(part 1 of 2)
# Autodesk Inventor assembly: Top_Backboard Assy
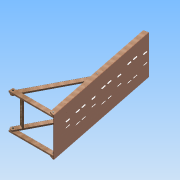
[picture p0: Inventor's stored thumbnail of the model, 180x180]
Saved by Autodesk Inventor 2018.1 (Build 221171000, 171)
## iProperties
Created: 2019-03-15
Part Number: Top_Backboard Assy
Document SubType Name: Assembly
Designer: James
Author: James
## Documents named in this file (20)
- C:\Users\admin\Desktop\Ball-Machine\Top Level\Top_Backboard Assy.iam
- C:\Users\admin\Desktop\Ball-Machine\Top Level\Top_Backboard.ipt
- C:\Users\admin\Desktop\Ball-Machine\Top Level\Top_Reinforcement 2.ipt
- C:\Users\admin\Desktop\Ball-Machine\Top Level\Top_Reinforcement_LHS.ipt
- C:\Users\admin\Desktop\Ball-Machine\Top Level\Top_Reinforcement_RHS.ipt
- C:\Users\admin\Desktop\Ball-Machine\Top Level\Din97 - 8x80 - Steel Wood Screw.ipt
- C:\Users\admin\Desktop\Ball-Machine\Top Level\Top_Hinge Cylinder.ipt
- C:\Users\admin\Desktop\Ball-Machine\Top Level\Top_Hinge End.ipt
- C:\Users\admin\Desktop\Ball-Machine\Top Level\Socket Cap Screw - Standard - (A2) - M8 x 20.ipt
- C:\Users\admin\Desktop\Ball-Machine\Top Level\Top_Floor Plank.ipt
- C:\Users\admin\Desktop\Ball-Machine\Top Level\Top_Reinforcement 3.ipt
- C:\Users\admin\Desktop\Ball-Machine\Top Level\Top_Rear Plank_RHS.ipt
- C:\Users\admin\Desktop\Ball-Machine\Top Level\Top_Rear Plank_LHS.ipt
- C:\Users\admin\Desktop\Ball-Machine\Top Level\Top_Spacer.ipt
- C:\Users\admin\Desktop\Ball-Machine\Top Level\Top_Hinge Cylinder Long.ipt
- C:\Users\admin\Desktop\Ball-Machine\Top Level\Top_Angle Bracket.ipt
- C:\Users\admin\Desktop\Ball-Machine\Selection Sort\Nyloc Nut - M4.ipt
- C:\Users\admin\Desktop\Ball-Machine\Selection Sort\Socket Cap Screw - Standard - (A2) - M4 x 16.ipt
- C:\Users\admin\Desktop\Ball-Machine\Top Level\Socket Cap Screw - Standard - (A2) - M4 x 25.ipt
- C:\Users\admin\Desktop\Ball-Machine\Top Level\Din97 - 4x25 - Steel Wood Screw.ipt
## Components (264 placed, 19 different names)
1. Top_Backboard:1 — Flush:3, Mate:1, Mate:2, Flush:5, Flush:6, Flush:7, Flush:8, Flush:10, Mate:5, Mate:320, Mate:321, Mate:322, Mate:323, Mate:324, Mate:325, Mate:326, Mate:327, Mate:328, Mate:329, Mate:330, Mate:331, Mate:332, Mate:333, Mate:334, Mate:335, Mate:336, Mate:337, Mate:338, Mate:339, Mate:340, Mate:341, Mate:342, Mate:343, Mate:344, Mate:345, Mate:346, Mate:347, Mate:348, Mate:349, Mate:350, Mate:351, Mate:352, Mate:353, Mate:354, Mate:355, Mate:356, Mate:357, Mate:358, Mate:359, Mate:360, Mate:361, Mate:362, Mate:363, Mate:364, Mate:365, Mate:366, Mate:367, Flush:29, Mate:368, Flush:30, Mate:369, Mate:370, Mate:371, Flush:31, Flush:32, Flush:33
2. Top_Reinforcement_LHS:1 — Mate:1, Flush:4, Flush:5, Flush:6, Flush:10, Mate:3, Mate:6, Mate:7, Mate:12, Mate:13, Flush:12, Mate:14, Mate:15, Mate:20, Mate:23, Mate:32, Mate:73, Mate:74, Mate:75, Mate:76, Mate:77, Mate:89, Mate:90, Mate:362
3. Top_Reinforcement_RHS:1 — Mate:2, Flush:4, Flush:7, Flush:8, Mate:4, Mate:8, Mate:9, Mate:10, Mate:11, Flush:13, Mate:21, Mate:22, Mate:31, Mate:55, Mate:56, Mate:64, Mate:65, Mate:66, Mate:67, Mate:68, Mate:82, Mate:83, Mate:363
4. Top_Floor Plank:1 — Mate:21, Mate:22, Flush:15, Mate:29, Mate:30, Mate:57, Mate:58, Mate:59
5. Top_Floor Plank:2 — Mate:20, Mate:23, Flush:15, Mate:24, Mate:25, Mate:26, Mate:27, Mate:28, Mate:61, Mate:62
6. Top_Rear Plank_RHS:1 — Mate:29, Mate:30, Flush:16, Mate:31, Mate:36, Mate:37, Mate:38, Mate:41, Mate:42, Flush:17, Mate:60, Mate:84, Mate:85
7. Top_Rear Plank_LHS:1 — Mate:27, Mate:28, Flush:16, Mate:32, Mate:33, Mate:34, Mate:35, Mate:39, Mate:40, Flush:20, Mate:63, Mate:91
8. Top_Reinforcement 3:1 — Mate:33, Mate:34, Mate:35, Mate:36, Mate:37, Mate:38
9. Top_Spacer:1 — Mate:64, Mate:65, Mate:66, Mate:67, Mate:68, Mate:69, Mate:70, Mate:71, Mate:72, Flush:24
10. Top_Spacer:2 — Mate:73, Mate:74, Mate:75, Mate:76, Mate:77, Flush:28, Mate:78, Mate:79, Mate:80, Mate:81
11. Top_Hinge End:6 — Mate:91, Mate:92, Mate:93, Mate:94, Mate:95
12. Top_Hinge Cylinder Long:2 — Mate:89, Mate:90, Mate:92, Mate:93
13. Din97 - 8x80 - Steel Wood Screw:17 — Mate:69, Flush:21
14. Din97 - 8x80 - Steel Wood Screw:18 — Mate:70, Flush:21, Flush:22, Flush:23, Flush:24
15. Din97 - 8x80 - Steel Wood Screw:19 — Mate:71, Flush:23
16. Din97 - 8x80 - Steel Wood Screw:20 — Mate:72, Flush:22
17. Din97 - 8x80 - Steel Wood Screw:21 — Flush:25, Flush:26, Flush:27, Flush:28, Mate:78
18. Din97 - 8x80 - Steel Wood Screw:22 — Flush:25, Mate:79
19. Din97 - 8x80 - Steel Wood Screw:23 — Flush:26, Mate:80
20. Din97 - 8x80 - Steel Wood Screw:24 — Flush:27, Mate:81
21. Socket Cap Screw - Standard - (A2) - M8 x 20:5 — Mate:87, Mate:88
22. Top_Hinge Cylinder Long:1 — Mate:82, Mate:83, Mate:86
23. Top_Hinge End:5 — Mate:84, Mate:85, Mate:86, Mate:87, Mate:88
24. Socket Cap Screw - Standard - (A2) - M8 x 20:6 — Mate:94, Mate:95
25. Socket Cap Screw - Standard - (A2) - M8 x 20:4
26. Top_Hinge End:4 — Mate:57
27. Top_Hinge Cylinder:4 — Mate:55, Mate:56
28. Socket Cap Screw - Standard - (A2) - M8 x 20:3
29. Top_Hinge End:3 — Mate:60
30. Top_Hinge Cylinder:3 — Mate:58, Mate:59
31. Socket Cap Screw - Standard - (A2) - M8 x 20:2
32. Top_Hinge End:2 — Mate:63
33. Top_Hinge Cylinder:2 — Mate:61, Mate:62
34. Din97 - 8x80 - Steel Wood Screw:16 — Mate:41, Flush:18
35. Din97 - 8x80 - Steel Wood Screw:15 — Mate:42, Flush:17, Flush:18
36. Din97 - 8x80 - Steel Wood Screw:14 — Mate:40, Flush:19, Flush:20
37. Din97 - 8x80 - Steel Wood Screw:13 — Mate:39, Flush:19
38. Socket Cap Screw - Standard - (A2) - M8 x 20:1 — Mate:18, Mate:19
39. Top_Hinge End:1 — Mate:16, Mate:17, Mate:18, Mate:19, Mate:26
40. Top_Hinge Cylinder:1 — Mate:14, Mate:15, Mate:16, Mate:17
41. Top_Angle Bracket:1 — Mate:104, Mate:105, Mate:106, Mate:107, Mate:108, Mate:109, Mate:110, Mate:111, Mate:320
42. Nyloc Nut - M4:1 — Mate:100
43. Nyloc Nut - M4:2 — Mate:103
44. Nyloc Nut - M4:3 — Mate:102
45. Socket Cap Screw - Standard - (A2) - M4 x 16:1 — Mate:102, Mate:108, Mate:110
46. Nyloc Nut - M4:4 — Mate:101
47. Socket Cap Screw - Standard - (A2) - M4 x 16:2 — Mate:101, Mate:109, Mate:111
48. Socket Cap Screw - Standard - (A2) - M4 x 25:1 — Mate:100, Mate:106, Mate:107, Mate:321
49. Socket Cap Screw - Standard - (A2) - M4 x 25:2 — Mate:103, Mate:104, Mate:105, Mate:322
50. Top_Angle Bracket:2 — Mate:323
51. Nyloc Nut - M4:5
52. Nyloc Nut - M4:6
53. Nyloc Nut - M4:7
54. Socket Cap Screw - Standard - (A2) - M4 x 16:3
55. Nyloc Nut - M4:8
56. Socket Cap Screw - Standard - (A2) - M4 x 16:4
57. Socket Cap Screw - Standard - (A2) - M4 x 25:3 — Mate:336
58. Socket Cap Screw - Standard - (A2) - M4 x 25:4 — Mate:337
59. Top_Angle Bracket:3 — Mate:324
60. Nyloc Nut - M4:9
61. Nyloc Nut - M4:10
62. Nyloc Nut - M4:11
63. Socket Cap Screw - Standard - (A2) - M4 x 16:5
64. Nyloc Nut - M4:12
65. Socket Cap Screw - Standard - (A2) - M4 x 16:6
66. Socket Cap Screw - Standard - (A2) - M4 x 25:5 — Mate:338
67. Socket Cap Screw - Standard - (A2) - M4 x 25:6 — Mate:339
68. Top_Angle Bracket:4 — Mate:325
69. Nyloc Nut - M4:13
70. Nyloc Nut - M4:14
71. Nyloc Nut - M4:15
72. Socket Cap Screw - Standard - (A2) - M4 x 16:7
73. Nyloc Nut - M4:16
74. Socket Cap Screw - Standard - (A2) - M4 x 16:8
75. Socket Cap Screw - Standard - (A2) - M4 x 25:7 — Mate:340
76. Socket Cap Screw - Standard - (A2) - M4 x 25:8 — Mate:341
77. Top_Angle Bracket:5 — Mate:326
78. Nyloc Nut - M4:17
79. Nyloc Nut - M4:18
80. Nyloc Nut - M4:19
81. Socket Cap Screw - Standard - (A2) - M4 x 16:9
82. Nyloc Nut - M4:20
83. Socket Cap Screw - Standard - (A2) - M4 x 16:10
84. Socket Cap Screw - Standard - (A2) - M4 x 25:9 — Mate:342
85. Socket Cap Screw - Standard - (A2) - M4 x 25:10 — Mate:343
86. Top_Angle Bracket:6 — Mate:327
87. Nyloc Nut - M4:21
88. Nyloc Nut - M4:22
89. Nyloc Nut - M4:23
90. Socket Cap Screw - Standard - (A2) - M4 x 16:11
91. Nyloc Nut - M4:24
92. Socket Cap Screw - Standard - (A2) - M4 x 16:12
93. Socket Cap Screw - Standard - (A2) - M4 x 25:11 — Mate:344
94. Socket Cap Screw - Standard - (A2) - M4 x 25:12 — Mate:345
95. Top_Angle Bracket:7 — Mate:328
96. Nyloc Nut - M4:25
97. Nyloc Nut - M4:26
98. Nyloc Nut - M4:27
99. Socket Cap Screw - Standard - (A2) - M4 x 16:13
100. Nyloc Nut - M4:28
101. Socket Cap Screw - Standard - (A2) - M4 x 16:14
102. Socket Cap Screw - Standard - (A2) - M4 x 25:13 — Mate:348
103. Socket Cap Screw - Standard - (A2) - M4 x 25:14 — Mate:349
104. Top_Angle Bracket:12 — Mate:333
105. Nyloc Nut - M4:45
106. Nyloc Nut - M4:46
107. Nyloc Nut - M4:47
108. Socket Cap Screw - Standard - (A2) - M4 x 16:23
109. Nyloc Nut - M4:48
110. Socket Cap Screw - Standard - (A2) - M4 x 16:24
111. Socket Cap Screw - Standard - (A2) - M4 x 25:23 — Mate:346
112. Socket Cap Screw - Standard - (A2) - M4 x 25:24 — Mate:347
113. Top_Reinforcement 2:1 — Mate:3, Mate:4, Mate:5, Mate:6, Mate:7, Mate:8, Mate:9, Mate:366
114. Din97 - 8x80 - Steel Wood Screw:1 — Mate:10, Flush:13, Flush:14
115. Din97 - 8x80 - Steel Wood Screw:2 — Mate:11, Flush:14
116. Din97 - 8x80 - Steel Wood Screw:3 — Mate:12, Flush:11, Flush:12
117. Din97 - 8x80 - Steel Wood Screw:4 — Mate:13, Flush:11
118. Top_Reinforcement 2:2 — Mate:364
119. Din97 - 8x80 - Steel Wood Screw:5
120. Din97 - 8x80 - Steel Wood Screw:6
121. Din97 - 8x80 - Steel Wood Screw:7
122. Din97 - 8x80 - Steel Wood Screw:8
123. Top_Reinforcement 2:3 — Mate:365
124. Din97 - 8x80 - Steel Wood Screw:9
125. Din97 - 8x80 - Steel Wood Screw:10
126. Din97 - 8x80 - Steel Wood Screw:11
127. Din97 - 8x80 - Steel Wood Screw:12
128. Top_Angle Bracket:14 — Mate:335
129. Socket Cap Screw - Standard - (A2) - M4 x 16:27
130. Socket Cap Screw - Standard - (A2) - M4 x 25:28 — Mate:361
131. Nyloc Nut - M4:55
132. Socket Cap Screw - Standard - (A2) - M4 x 16:28
133. Socket Cap Screw - Standard - (A2) - M4 x 25:27 — Mate:360
134. Nyloc Nut - M4:56
135. Nyloc Nut - M4:52
136. Socket Cap Screw - Standard - (A2) - M4 x 16:26
137. Socket Cap Screw - Standard - (A2) - M4 x 25:25 — Mate:358
138. Top_Angle Bracket:13 — Mate:334
139. Nyloc Nut - M4:51
140. Socket Cap Screw - Standard - (A2) - M4 x 16:25
141. Socket Cap Screw - Standard - (A2) - M4 x 25:26 — Mate:359
142. Socket Cap Screw - Standard - (A2) - M4 x 25:18 — Mate:353
143. Socket Cap Screw - Standard - (A2) - M4 x 16:17
144. Top_Angle Bracket:9 — Mate:330
145. Nyloc Nut - M4:35
146. Socket Cap Screw - Standard - (A2) - M4 x 25:17 — Mate:352
147. Socket Cap Screw - Standard - (A2) - M4 x 16:18
148. Nyloc Nut - M4:36
149. Nyloc Nut - M4:32
150. Socket Cap Screw - Standard - (A2) - M4 x 16:16
151. Socket Cap Screw - Standard - (A2) - M4 x 25:15 — Mate:350
152. Top_Angle Bracket:8 — Mate:329
153. Nyloc Nut - M4:31
154. Socket Cap Screw - Standard - (A2) - M4 x 16:15
155. Socket Cap Screw - Standard - (A2) - M4 x 25:16 — Mate:351
156. Socket Cap Screw - Standard - (A2) - M4 x 25:22 — Mate:357
157. Socket Cap Screw - Standard - (A2) - M4 x 16:21
158. Top_Angle Bracket:11 — Mate:332
159. Nyloc Nut - M4:43
160. Socket Cap Screw - Standard - (A2) - M4 x 25:21 — Mate:356
161. Socket Cap Screw - Standard - (A2) - M4 x 16:22
162. Nyloc Nut - M4:44
163. Nyloc Nut - M4:40
164. Socket Cap Screw - Standard - (A2) - M4 x 16:20
165. Top_Angle Bracket:10 — Mate:331
166. Socket Cap Screw - Standard - (A2) - M4 x 25:19 — Mate:354
167. Nyloc Nut - M4:39
168. Socket Cap Screw - Standard - (A2) - M4 x 16:19
169. Socket Cap Screw - Standard - (A2) - M4 x 25:20 — Mate:355
170. Nyloc Nut - M4:37
171. Nyloc Nut - M4:38
172. Nyloc Nut - M4:41
173. Nyloc Nut - M4:42
174. Nyloc Nut - M4:33
175. Nyloc Nut - M4:34
176. Nyloc Nut - M4:29
177. Nyloc Nut - M4:30
178. Nyloc Nut - M4:53
179. Nyloc Nut - M4:54
180. Nyloc Nut - M4:49
181. Nyloc Nut - M4:50
182. Top_Angle Bracket:15
183. Socket Cap Screw - Standard - (A2) - M4 x 16:29
184. Socket Cap Screw - Standard - (A2) - M4 x 25:29
185. Nyloc Nut - M4:57
186. Socket Cap Screw - Standard - (A2) - M4 x 16:30
187. Socket Cap Screw - Standard - (A2) - M4 x 25:30
188. Nyloc Nut - M4:58
189. Nyloc Nut - M4:59
190. Socket Cap Screw - Standard - (A2) - M4 x 16:31
191. Socket Cap Screw - Standard - (A2) - M4 x 25:31
192. Top_Angle Bracket:16
193. Nyloc Nut - M4:60
194. Socket Cap Screw - Standard - (A2) - M4 x 16:32
195. Socket Cap Screw - Standard - (A2) - M4 x 25:32
196. Socket Cap Screw - Standard - (A2) - M4 x 25:33
197. Socket Cap Screw - Standard - (A2) - M4 x 16:33
198. Top_Angle Bracket:17
199. Nyloc Nut - M4:61
200. Socket Cap Screw - Standard - (A2) - M4 x 25:34
201. Socket Cap Screw - Standard - (A2) - M4 x 16:34
202. Nyloc Nut - M4:62
203. Nyloc Nut - M4:63
204. Socket Cap Screw - Standard - (A2) - M4 x 16:35
205. Socket Cap Screw - Standard - (A2) - M4 x 25:35
206. Top_Angle Bracket:18
207. Nyloc Nut - M4:64
208. Socket Cap Screw - Standard - (A2) - M4 x 16:36
209. Socket Cap Screw - Standard - (A2) - M4 x 25:36
210. Socket Cap Screw - Standard - (A2) - M4 x 25:37
211. Socket Cap Screw - Standard - (A2) - M4 x 16:37
212. Top_Angle Bracket:19
213. Nyloc Nut - M4:65
214. Socket Cap Screw - Standard - (A2) - M4 x 25:38
215. Socket Cap Screw - Standard - (A2) - M4 x 16:38
216. Nyloc Nut - M4:66
217. Nyloc Nut - M4:67
218. Socket Cap Screw - Standard - (A2) - M4 x 16:39
219. Top_Angle Bracket:20
220. Socket Cap Screw - Standard - (A2) - M4 x 25:39
221. Nyloc Nut - M4:68
222. Socket Cap Screw - Standard - (A2) - M4 x 16:40
223. Socket Cap Screw - Standard - (A2) - M4 x 25:40
224. Nyloc Nut - M4:69
225. Nyloc Nut - M4:70
226. Nyloc Nut - M4:71
227. Nyloc Nut - M4:72
228. Nyloc Nut - M4:73
229. Nyloc Nut - M4:74
230. Nyloc Nut - M4:75
231. Nyloc Nut - M4:76
232. Nyloc Nut - M4:77
233. Nyloc Nut - M4:78
234. Nyloc Nut - M4:79
235. Nyloc Nut - M4:80
236. Din97 - 4x25 - Steel Wood Screw:1 — Mate:367, Flush:29
237. Din97 - 4x25 - Steel Wood Screw:2 — Mate:368, Flush:30
238. Din97 - 4x25 - Steel Wood Screw:6
239. Din97 - 4x25 - Steel Wood Screw:7
240. Din97 - 4x25 - Steel Wood Screw:8
241. Din97 - 4x25 - Steel Wood Screw:9
242. Din97 - 4x25 - Steel Wood Screw:10
243. Din97 - 4x25 - Steel Wood Screw:11
244. Din97 - 4x25 - Steel Wood Screw:12
245. Din97 - 4x25 - Steel Wood Screw:13
246. Din97 - 4x25 - Steel Wood Screw:14
247. Din97 - 4x25 - Steel Wood Screw:15
248. Din97 - 4x25 - Steel Wood Screw:16
249. Din97 - 4x25 - Steel Wood Screw:17
250. Din97 - 4x25 - Steel Wood Screw:18
251. Din97 - 4x25 - Steel Wood Screw:19
252. Din97 - 4x25 - Steel Wood Screw:20
253. Din97 - 4x25 - Steel Wood Screw:21
254. Din97 - 4x25 - Steel Wood Screw:22
255. Din97 - 4x25 - Steel Wood Screw:23
256. Din97 - 4x25 - Steel Wood Screw:3 — Mate:369, Flush:31
257. Din97 - 4x25 - Steel Wood Screw:4 — Mate:371, Flush:32
258. Din97 - 4x25 - Steel Wood Screw:5 — Mate:370, Flush:33
259. Din97 - 4x25 - Steel Wood Screw:24
260. Din97 - 4x25 - Steel Wood Screw:25
261. Din97 - 4x25 - Steel Wood Screw:26
262. Din97 - 4x25 - Steel Wood Screw:27
263. Din97 - 4x25 - Steel Wood Screw:28
264. Din97 - 4x25 - Steel Wood Screw:29
## Component patterns: (3 elements, first: Top_Reinforcement 2:1 + Din97 - 8x80 - Steel Wood Screw:1 + Din97 - 8x80 - Steel Wood Screw:2 + Din97 - 8x80 - Steel Wood Screw:3 + Din97 - 8x80 - Steel Wood Screw:4), (2 elements, first: Top_Angle Bracket:14 + Socket Cap Screw - Standard - (A2) - M4 x 16:27 + Socket Cap Screw - Standard - (A2) - M4 x 25:28 + Nyloc Nut - M4:55 + Socket Cap Screw - Standard - (A2) - M4 x 16:28 + Socket Cap Screw - Standard - (A2) - M4 x 25:27 + Nyloc Nut - M4:56 + Nyloc Nut - M4:52 + Socket Cap Screw - Standard - (A2) - M4 x 16:26 + Socket Cap Screw - Standard - (A2) - M4 x 25:25 + Top_Angle Bracket:13 + Nyloc Nut - M4:51 + Socket Cap Screw - Standard - (A2) - M4 x 16:25 + Socket Cap Screw - Standard - (A2) - M4 x 25:26 + Socket Cap Screw - Standard - (A2) - M4 x 25:18 + Socket Cap Screw - Standard - (A2) - M4 x 16:17 + Top_Angle Bracket:9 + Nyloc Nut - M4:35 + Socket Cap Screw - Standard - (A2) - M4 x 25:17 + Socket Cap Screw - Standard - (A2) - M4 x 16:18 + Nyloc Nut - M4:36 + Nyloc Nut - M4:32 + Socket Cap Screw - Standard - (A2) - M4 x 16:16 + Socket Cap Screw - Standard - (A2) - M4 x 25:15 + Top_Angle Bracket:8 + Nyloc Nut - M4:31 + Socket Cap Screw - Standard - (A2) - M4 x 16:15 + Socket Cap Screw - Standard - (A2) - M4 x 25:16 + Socket Cap Screw - Standard - (A2) - M4 x 25:22 + Socket Cap Screw - Standard - (A2) - M4 x 16:21 + Top_Angle Bracket:11 + Nyloc Nut - M4:43 + Socket Cap Screw - Standard - (A2) - M4 x 25:21 + Socket Cap Screw - Standard - (A2) - M4 x 16:22 + Nyloc Nut - M4:44 + Nyloc Nut - M4:40 + Socket Cap Screw - Standard - (A2) - M4 x 16:20 + Top_Angle Bracket:10 + Socket Cap Screw - Standard - (A2) - M4 x 25:19 + Nyloc Nut - M4:39 + Socket Cap Screw - Standard - (A2) - M4 x 16:19 + Socket Cap Screw - Standard - (A2) - M4 x 25:20 + Nyloc Nut - M4:37 + Nyloc Nut - M4:38 + Nyloc Nut - M4:41 + Nyloc Nut - M4:42 + Nyloc Nut - M4:33 + Nyloc Nut - M4:34 + Nyloc Nut - M4:29 + Nyloc Nut - M4:30 + Nyloc Nut - M4:53 + Nyloc Nut - M4:54 + Nyloc Nut - M4:49 + Nyloc Nut - M4:50), (10 elements, first: Din97 - 4x25 - Steel Wood Screw:1 + Din97 - 4x25 - Steel Wood Screw:2), (3 elements, first: Din97 - 4x25 - Steel Wood Screw:3 + Din97 - 4x25 - Steel Wood Screw:4 + Din97 - 4x25 - Steel Wood Screw:5)
## Relationships (401: Mate 371, Flush 30)
- Flush:3: Top_Backboard:1
- Mate:1: Top_Backboard:1 ↔ Top_Reinforcement_LHS:1
- Mate:2: Top_Backboard:1 ↔ Top_Reinforcement_RHS:1
- Flush:4: Top_Reinforcement_LHS:1 ↔ Top_Reinforcement_RHS:1
- Flush:5: Top_Backboard:1 ↔ Top_Reinforcement_LHS:1
- Flush:6: Top_Backboard:1 ↔ Top_Reinforcement_LHS:1
- Flush:7: Top_Backboard:1 ↔ Top_Reinforcement_RHS:1
- Flush:8: Top_Backboard:1 ↔ Top_Reinforcement_RHS:1
- Flush:10: Top_Backboard:1 ↔ Top_Reinforcement_LHS:1
- Mate:3: Top_Reinforcement_LHS:1 ↔ Top_Reinforcement 2:1
- Mate:4: Top_Reinforcement_RHS:1 ↔ Top_Reinforcement 2:1
- Mate:5: Top_Backboard:1 ↔ Top_Reinforcement 2:1
- Mate:6: Top_Reinforcement_LHS:1 ↔ Top_Reinforcement 2:1
- Mate:7: Top_Reinforcement_LHS:1 ↔ Top_Reinforcement 2:1
- Mate:8: Top_Reinforcement_RHS:1 ↔ Top_Reinforcement 2:1
- Mate:9: Top_Reinforcement_RHS:1 ↔ Top_Reinforcement 2:1
- Mate:10: Top_Reinforcement_RHS:1 ↔ Din97 - 8x80 - Steel Wood Screw:1
- Mate:11: Top_Reinforcement_RHS:1 ↔ Din97 - 8x80 - Steel Wood Screw:2
- Mate:12: Top_Reinforcement_LHS:1 ↔ Din97 - 8x80 - Steel Wood Screw:3
- Mate:13: Top_Reinforcement_LHS:1 ↔ Din97 - 8x80 - Steel Wood Screw:4
- Flush:11: Din97 - 8x80 - Steel Wood Screw:3 ↔ Din97 - 8x80 - Steel Wood Screw:4
- Flush:12: Top_Reinforcement_LHS:1 ↔ Din97 - 8x80 - Steel Wood Screw:3
- Flush:13: Top_Reinforcement_RHS:1 ↔ Din97 - 8x80 - Steel Wood Screw:1
- Flush:14: Din97 - 8x80 - Steel Wood Screw:1 ↔ Din97 - 8x80 - Steel Wood Screw:2
- Mate:14: Top_Reinforcement_LHS:1 ↔ Top_Hinge Cylinder:1
- Mate:15: Top_Reinforcement_LHS:1 ↔ Top_Hinge Cylinder:1
- Mate:16: Top_Hinge End:1 ↔ Top_Hinge Cylinder:1
- Mate:17: Top_Hinge End:1 ↔ Top_Hinge Cylinder:1
- Mate:18: Socket Cap Screw - Standard - (A2) - M8 x 20:1 ↔ Top_Hinge End:1
- Mate:19: Socket Cap Screw - Standard - (A2) - M8 x 20:1 ↔ Top_Hinge End:1
- Mate:20: Top_Reinforcement_LHS:1 ↔ Top_Floor Plank:2
- Mate:21: Top_Reinforcement_RHS:1 ↔ Top_Floor Plank:1
- Mate:22: Top_Reinforcement_RHS:1 ↔ Top_Floor Plank:1
- Mate:23: Top_Reinforcement_LHS:1 ↔ Top_Floor Plank:2
- Flush:15: Top_Floor Plank:1 ↔ Top_Floor Plank:2
- Mate:24: Top_Floor Plank:2
- Mate:25: Top_Floor Plank:2
- Mate:26: Top_Floor Plank:2 ↔ Top_Hinge End:1
- Mate:27: Top_Floor Plank:2 ↔ Top_Rear Plank_LHS:1
- Mate:28: Top_Floor Plank:2 ↔ Top_Rear Plank_LHS:1
- Mate:29: Top_Floor Plank:1 ↔ Top_Rear Plank_RHS:1
- Mate:30: Top_Floor Plank:1 ↔ Top_Rear Plank_RHS:1
- Flush:16: Top_Rear Plank_RHS:1 ↔ Top_Rear Plank_LHS:1
- Mate:31: Top_Reinforcement_RHS:1 ↔ Top_Rear Plank_RHS:1
- Mate:32: Top_Reinforcement_LHS:1 ↔ Top_Rear Plank_LHS:1
- Mate:33: Top_Rear Plank_LHS:1 ↔ Top_Reinforcement 3:1
- Mate:34: Top_Rear Plank_LHS:1 ↔ Top_Reinforcement 3:1
- Mate:35: Top_Rear Plank_LHS:1 ↔ Top_Reinforcement 3:1
- Mate:36: Top_Rear Plank_RHS:1 ↔ Top_Reinforcement 3:1
- Mate:37: Top_Rear Plank_RHS:1 ↔ Top_Reinforcement 3:1
- Mate:38: Top_Rear Plank_RHS:1 ↔ Top_Reinforcement 3:1
- Mate:39: Top_Rear Plank_LHS:1 ↔ Din97 - 8x80 - Steel Wood Screw:13
- Mate:40: Top_Rear Plank_LHS:1 ↔ Din97 - 8x80 - Steel Wood Screw:14
- Mate:41: Top_Rear Plank_RHS:1 ↔ Din97 - 8x80 - Steel Wood Screw:16
- Mate:42: Top_Rear Plank_RHS:1 ↔ Din97 - 8x80 - Steel Wood Screw:15
- Flush:17: Top_Rear Plank_RHS:1 ↔ Din97 - 8x80 - Steel Wood Screw:15
- Flush:18: Din97 - 8x80 - Steel Wood Screw:16 ↔ Din97 - 8x80 - Steel Wood Screw:15
- Flush:19: Din97 - 8x80 - Steel Wood Screw:14 ↔ Din97 - 8x80 - Steel Wood Screw:13
- Flush:20: Top_Rear Plank_LHS:1 ↔ Din97 - 8x80 - Steel Wood Screw:14
- [Mate]: Top_Hinge End:2 ↔ Top_Hinge Cylinder:2
- [Mate]: Top_Hinge End:2 ↔ Top_Hinge Cylinder:2
- [Mate]: Socket Cap Screw - Standard - (A2) - M8 x 20:2 ↔ Top_Hinge End:2
- [Mate]: Socket Cap Screw - Standard - (A2) - M8 x 20:2 ↔ Top_Hinge End:2
- [Mate]: Top_Hinge End:3 ↔ Top_Hinge Cylinder:3
- [Mate]: Top_Hinge End:3 ↔ Top_Hinge Cylinder:3
- [Mate]: Socket Cap Screw - Standard - (A2) - M8 x 20:3 ↔ Top_Hinge End:3
- [Mate]: Socket Cap Screw - Standard - (A2) - M8 x 20:3 ↔ Top_Hinge End:3
- [Mate]: Top_Hinge End:4 ↔ Top_Hinge Cylinder:4
- [Mate]: Top_Hinge End:4 ↔ Top_Hinge Cylinder:4
- [Mate]: Socket Cap Screw - Standard - (A2) - M8 x 20:4 ↔ Top_Hinge End:4
- [Mate]: Socket Cap Screw - Standard - (A2) - M8 x 20:4 ↔ Top_Hinge End:4
- Mate:55: Top_Reinforcement_RHS:1 ↔ Top_Hinge Cylinder:4
- Mate:56: Top_Reinforcement_RHS:1 ↔ Top_Hinge Cylinder:4
- Mate:57: Top_Floor Plank:1 ↔ Top_Hinge End:4
- Mate:58: Top_Floor Plank:1 ↔ Top_Hinge Cylinder:3
- Mate:59: Top_Floor Plank:1 ↔ Top_Hinge Cylinder:3
- Mate:60: Top_Rear Plank_RHS:1 ↔ Top_Hinge End:3
- Mate:61: Top_Floor Plank:2 ↔ Top_Hinge Cylinder:2
- Mate:62: Top_Floor Plank:2 ↔ Top_Hinge Cylinder:2
- Mate:63: Top_Rear Plank_LHS:1 ↔ Top_Hinge End:2
- Mate:64: Top_Reinforcement_RHS:1 ↔ Top_Spacer:1
- Mate:65: Top_Reinforcement_RHS:1 ↔ Top_Spacer:1
- Mate:66: Top_Reinforcement_RHS:1 ↔ Top_Spacer:1
- Mate:67: Top_Reinforcement_RHS:1 ↔ Top_Spacer:1
- Mate:68: Top_Reinforcement_RHS:1 ↔ Top_Spacer:1
- Mate:69: Top_Spacer:1 ↔ Din97 - 8x80 - Steel Wood Screw:17
- Mate:70: Top_Spacer:1 ↔ Din97 - 8x80 - Steel Wood Screw:18
- Mate:71: Top_Spacer:1 ↔ Din97 - 8x80 - Steel Wood Screw:19
- Mate:72: Top_Spacer:1 ↔ Din97 - 8x80 - Steel Wood Screw:20
- Flush:21: Din97 - 8x80 - Steel Wood Screw:17 ↔ Din97 - 8x80 - Steel Wood Screw:18
- Flush:22: Din97 - 8x80 - Steel Wood Screw:18 ↔ Din97 - 8x80 - Steel Wood Screw:20
- Flush:23: Din97 - 8x80 - Steel Wood Screw:18 ↔ Din97 - 8x80 - Steel Wood Screw:19
- Flush:24: Top_Spacer:1 ↔ Din97 - 8x80 - Steel Wood Screw:18
- Mate:73: Top_Reinforcement_LHS:1 ↔ Top_Spacer:2
- Mate:74: Top_Reinforcement_LHS:1 ↔ Top_Spacer:2
- Mate:75: Top_Reinforcement_LHS:1 ↔ Top_Spacer:2
- Mate:76: Top_Reinforcement_LHS:1 ↔ Top_Spacer:2
- Mate:77: Top_Reinforcement_LHS:1 ↔ Top_Spacer:2
- Flush:25: Din97 - 8x80 - Steel Wood Screw:21 ↔ Din97 - 8x80 - Steel Wood Screw:22
- Flush:26: Din97 - 8x80 - Steel Wood Screw:21 ↔ Din97 - 8x80 - Steel Wood Screw:23
- Flush:27: Din97 - 8x80 - Steel Wood Screw:21 ↔ Din97 - 8x80 - Steel Wood Screw:24
- Flush:28: Top_Spacer:2 ↔ Din97 - 8x80 - Steel Wood Screw:21
- Mate:78: Top_Spacer:2 ↔ Din97 - 8x80 - Steel Wood Screw:21
- Mate:79: Top_Spacer:2 ↔ Din97 - 8x80 - Steel Wood Screw:22
- Mate:80: Top_Spacer:2 ↔ Din97 - 8x80 - Steel Wood Screw:23
- Mate:81: Top_Spacer:2 ↔ Din97 - 8x80 - Steel Wood Screw:24
- Mate:82: Top_Reinforcement_RHS:1 ↔ Top_Hinge Cylinder Long:1
- Mate:83: Top_Reinforcement_RHS:1 ↔ Top_Hinge Cylinder Long:1
- Mate:84: Top_Rear Plank_RHS:1 ↔ Top_Hinge End:5
- Mate:85: Top_Rear Plank_RHS:1 ↔ Top_Hinge End:5
- Mate:86: Top_Hinge Cylinder Long:1 ↔ Top_Hinge End:5
- Mate:87: Socket Cap Screw - Standard - (A2) - M8 x 20:5 ↔ Top_Hinge End:5
- Mate:88: Socket Cap Screw - Standard - (A2) - M8 x 20:5 ↔ Top_Hinge End:5
- Mate:89: Top_Reinforcement_LHS:1 ↔ Top_Hinge Cylinder Long:2
- Mate:90: Top_Reinforcement_LHS:1 ↔ Top_Hinge Cylinder Long:2
- Mate:91: Top_Rear Plank_LHS:1 ↔ Top_Hinge End:6
- Mate:92: Top_Hinge End:6 ↔ Top_Hinge Cylinder Long:2
- Mate:93: Top_Hinge End:6 ↔ Top_Hinge Cylinder Long:2
- Mate:94: Top_Hinge End:6 ↔ Socket Cap Screw - Standard - (A2) - M8 x 20:6
- Mate:95: Top_Hinge End:6 ↔ Socket Cap Screw - Standard - (A2) - M8 x 20:6
- [Mate]: Nyloc Nut - M4:1 ↔ Socket Cap Screw - Standard - (A2) - M4 x 25:1
- [Mate]: Nyloc Nut - M4:2 ↔ Socket Cap Screw - Standard - (A2) - M4 x 25:2
- [Mate]: Nyloc Nut - M4:3 ↔ Socket Cap Screw - Standard - (A2) - M4 x 16:1
- [Mate]: Nyloc Nut - M4:4 ↔ Socket Cap Screw - Standard - (A2) - M4 x 16:2
- Mate:100 (18 mm): Nyloc Nut - M4:1 ↔ Socket Cap Screw - Standard - (A2) - M4 x 25:1
- Mate:101 (8 mm): Nyloc Nut - M4:4 ↔ Socket Cap Screw - Standard - (A2) - M4 x 16:2
- Mate:102 (8 mm): Nyloc Nut - M4:3 ↔ Socket Cap Screw - Standard - (A2) - M4 x 16:1
- Mate:103 (18 mm): Nyloc Nut - M4:2 ↔ Socket Cap Screw - Standard - (A2) - M4 x 25:2
- Mate:104: Top_Angle Bracket:1 ↔ Socket Cap Screw - Standard - (A2) - M4 x 25:2
- Mate:105: Top_Angle Bracket:1 ↔ Socket Cap Screw - Standard - (A2) - M4 x 25:2
- Mate:106: Top_Angle Bracket:1 ↔ Socket Cap Screw - Standard - (A2) - M4 x 25:1
- Mate:107: Top_Angle Bracket:1 ↔ Socket Cap Screw - Standard - (A2) - M4 x 25:1
- Mate:108: Top_Angle Bracket:1 ↔ Socket Cap Screw - Standard - (A2) - M4 x 16:1
- Mate:109: Top_Angle Bracket:1 ↔ Socket Cap Screw - Standard - (A2) - M4 x 16:2
- Mate:110: Top_Angle Bracket:1 ↔ Socket Cap Screw - Standard - (A2) - M4 x 16:1
- Mate:111: Top_Angle Bracket:1 ↔ Socket Cap Screw - Standard - (A2) - M4 x 16:2
- [Mate]: Nyloc Nut - M4:5 ↔ Socket Cap Screw - Standard - (A2) - M4 x 25:3
- [Mate]: Nyloc Nut - M4:6 ↔ Socket Cap Screw - Standard - (A2) - M4 x 25:4
- [Mate]: Nyloc Nut - M4:7 ↔ Socket Cap Screw - Standard - (A2) - M4 x 16:3
- [Mate]: Nyloc Nut - M4:8 ↔ Socket Cap Screw - Standard - (A2) - M4 x 16:4
- [Mate] (18 mm): Nyloc Nut - M4:5 ↔ Socket Cap Screw - Standard - (A2) - M4 x 25:3
- [Mate] (8 mm): Nyloc Nut - M4:8 ↔ Socket Cap Screw - Standard - (A2) - M4 x 16:4
- [Mate] (8 mm): Nyloc Nut - M4:7 ↔ Socket Cap Screw - Standard - (A2) - M4 x 16:3
- [Mate] (18 mm): Nyloc Nut - M4:6 ↔ Socket Cap Screw - Standard - (A2) - M4 x 25:4
- [Mate]: Top_Angle Bracket:2 ↔ Socket Cap Screw - Standard - (A2) - M4 x 25:4
- [Mate]: Top_Angle Bracket:2 ↔ Socket Cap Screw - Standard - (A2) - M4 x 25:4
- [Mate]: Top_Angle Bracket:2 ↔ Socket Cap Screw - Standard - (A2) - M4 x 25:3
- [Mate]: Top_Angle Bracket:2 ↔ Socket Cap Screw - Standard - (A2) - M4 x 25:3
- [Mate]: Top_Angle Bracket:2 ↔ Socket Cap Screw - Standard - (A2) - M4 x 16:3
- [Mate]: Top_Angle Bracket:2 ↔ Socket Cap Screw - Standard - (A2) - M4 x 16:4
- [Mate]: Top_Angle Bracket:2 ↔ Socket Cap Screw - Standard - (A2) - M4 x 16:3
- [Mate]: Top_Angle Bracket:2 ↔ Socket Cap Screw - Standard - (A2) - M4 x 16:4
- [Mate]: Nyloc Nut - M4:9 ↔ Socket Cap Screw - Standard - (A2) - M4 x 25:5
- [Mate]: Nyloc Nut - M4:10 ↔ Socket Cap Screw - Standard - (A2) - M4 x 25:6
- [Mate]: Nyloc Nut - M4:11 ↔ Socket Cap Screw - Standard - (A2) - M4 x 16:5
- [Mate]: Nyloc Nut - M4:12 ↔ Socket Cap Screw - Standard - (A2) - M4 x 16:6
- [Mate] (18 mm): Nyloc Nut - M4:9 ↔ Socket Cap Screw - Standard - (A2) - M4 x 25:5
- [Mate] (8 mm): Nyloc Nut - M4:12 ↔ Socket Cap Screw - Standard - (A2) - M4 x 16:6
- [Mate] (8 mm): Nyloc Nut - M4:11 ↔ Socket Cap Screw - Standard - (A2) - M4 x 16:5
- [Mate] (18 mm): Nyloc Nut - M4:10 ↔ Socket Cap Screw - Standard - (A2) - M4 x 25:6
- [Mate]: Top_Angle Bracket:3 ↔ Socket Cap Screw - Standard - (A2) - M4 x 25:6
- [Mate]: Top_Angle Bracket:3 ↔ Socket Cap Screw - Standard - (A2) - M4 x 25:6
- [Mate]: Top_Angle Bracket:3 ↔ Socket Cap Screw - Standard - (A2) - M4 x 25:5
- [Mate]: Top_Angle Bracket:3 ↔ Socket Cap Screw - Standard - (A2) - M4 x 25:5
- [Mate]: Top_Angle Bracket:3 ↔ Socket Cap Screw - Standard - (A2) - M4 x 16:5
- [Mate]: Top_Angle Bracket:3 ↔ Socket Cap Screw - Standard - (A2) - M4 x 16:6
- [Mate]: Top_Angle Bracket:3 ↔ Socket Cap Screw - Standard - (A2) - M4 x 16:5
- [Mate]: Top_Angle Bracket:3 ↔ Socket Cap Screw - Standard - (A2) - M4 x 16:6
- [Mate]: Nyloc Nut - M4:13 ↔ Socket Cap Screw - Standard - (A2) - M4 x 25:7
- [Mate]: Nyloc Nut - M4:14 ↔ Socket Cap Screw - Standard - (A2) - M4 x 25:8
- [Mate]: Nyloc Nut - M4:15 ↔ Socket Cap Screw - Standard - (A2) - M4 x 16:7
- [Mate]: Nyloc Nut - M4:16 ↔ Socket Cap Screw - Standard - (A2) - M4 x 16:8
- [Mate] (18 mm): Nyloc Nut - M4:13 ↔ Socket Cap Screw - Standard - (A2) - M4 x 25:7
- [Mate] (8 mm): Nyloc Nut - M4:16 ↔ Socket Cap Screw - Standard - (A2) - M4 x 16:8
- [Mate] (8 mm): Nyloc Nut - M4:15 ↔ Socket Cap Screw - Standard - (A2) - M4 x 16:7
- [Mate] (18 mm): Nyloc Nut - M4:14 ↔ Socket Cap Screw - Standard - (A2) - M4 x 25:8
- [Mate]: Top_Angle Bracket:4 ↔ Socket Cap Screw - Standard - (A2) - M4 x 25:8
- [Mate]: Top_Angle Bracket:4 ↔ Socket Cap Screw - Standard - (A2) - M4 x 25:8
- [Mate]: Top_Angle Bracket:4 ↔ Socket Cap Screw - Standard - (A2) - M4 x 25:7
- [Mate]: Top_Angle Bracket:4 ↔ Socket Cap Screw - Standard - (A2) - M4 x 25:7
- [Mate]: Top_Angle Bracket:4 ↔ Socket Cap Screw - Standard - (A2) - M4 x 16:7
- [Mate]: Top_Angle Bracket:4 ↔ Socket Cap Screw - Standard - (A2) - M4 x 16:8
- [Mate]: Top_Angle Bracket:4 ↔ Socket Cap Screw - Standard - (A2) - M4 x 16:7
- [Mate]: Top_Angle Bracket:4 ↔ Socket Cap Screw - Standard - (A2) - M4 x 16:8
- [Mate]: Nyloc Nut - M4:17 ↔ Socket Cap Screw - Standard - (A2) - M4 x 25:9
- [Mate]: Nyloc Nut - M4:18 ↔ Socket Cap Screw - Standard - (A2) - M4 x 25:10
- [Mate]: Nyloc Nut - M4:19 ↔ Socket Cap Screw - Standard - (A2) - M4 x 16:9
- [Mate]: Nyloc Nut - M4:20 ↔ Socket Cap Screw - Standard - (A2) - M4 x 16:10
- [Mate] (18 mm): Nyloc Nut - M4:17 ↔ Socket Cap Screw - Standard - (A2) - M4 x 25:9
- [Mate] (8 mm): Nyloc Nut - M4:20 ↔ Socket Cap Screw - Standard - (A2) - M4 x 16:10
- [Mate] (8 mm): Nyloc Nut - M4:19 ↔ Socket Cap Screw - Standard - (A2) - M4 x 16:9
- [Mate] (18 mm): Nyloc Nut - M4:18 ↔ Socket Cap Screw - Standard - (A2) - M4 x 25:10
- [Mate]: Top_Angle Bracket:5 ↔ Socket Cap Screw - Standard - (A2) - M4 x 25:10
- [Mate]: Top_Angle Bracket:5 ↔ Socket Cap Screw - Standard - (A2) - M4 x 25:10
- [Mate]: Top_Angle Bracket:5 ↔ Socket Cap Screw - Standard - (A2) - M4 x 25:9
- [Mate]: Top_Angle Bracket:5 ↔ Socket Cap Screw - Standard - (A2) - M4 x 25:9
- [Mate]: Top_Angle Bracket:5 ↔ Socket Cap Screw - Standard - (A2) - M4 x 16:9
- [Mate]: Top_Angle Bracket:5 ↔ Socket Cap Screw - Standard - (A2) - M4 x 16:10
- [Mate]: Top_Angle Bracket:5 ↔ Socket Cap Screw - Standard - (A2) - M4 x 16:9
- [Mate]: Top_Angle Bracket:5 ↔ Socket Cap Screw - Standard - (A2) - M4 x 16:10
- [Mate]: Nyloc Nut - M4:21 ↔ Socket Cap Screw - Standard - (A2) - M4 x 25:11
- [Mate]: Nyloc Nut - M4:22 ↔ Socket Cap Screw - Standard - (A2) - M4 x 25:12
- [Mate]: Nyloc Nut - M4:23 ↔ Socket Cap Screw - Standard - (A2) - M4 x 16:11
- [Mate]: Nyloc Nut - M4:24 ↔ Socket Cap Screw - Standard - (A2) - M4 x 16:12
- [Mate] (18 mm): Nyloc Nut - M4:21 ↔ Socket Cap Screw - Standard - (A2) - M4 x 25:11
- [Mate] (8 mm): Nyloc Nut - M4:24 ↔ Socket Cap Screw - Standard - (A2) - M4 x 16:12
- [Mate] (8 mm): Nyloc Nut - M4:23 ↔ Socket Cap Screw - Standard - (A2) - M4 x 16:11
- [Mate] (18 mm): Nyloc Nut - M4:22 ↔ Socket Cap Screw - Standard - (A2) - M4 x 25:12
- [Mate]: Top_Angle Bracket:6 ↔ Socket Cap Screw - Standard - (A2) - M4 x 25:12
- [Mate]: Top_Angle Bracket:6 ↔ Socket Cap Screw - Standard - (A2) - M4 x 25:12
- [Mate]: Top_Angle Bracket:6 ↔ Socket Cap Screw - Standard - (A2) - M4 x 25:11
- [Mate]: Top_Angle Bracket:6 ↔ Socket Cap Screw - Standard - (A2) - M4 x 25:11
- [Mate]: Top_Angle Bracket:6 ↔ Socket Cap Screw - Standard - (A2) - M4 x 16:11
- [Mate]: Top_Angle Bracket:6 ↔ Socket Cap Screw - Standard - (A2) - M4 x 16:12
- [Mate]: Top_Angle Bracket:6 ↔ Socket Cap Screw - Standard - (A2) - M4 x 16:11
- [Mate]: Top_Angle Bracket:6 ↔ Socket Cap Screw - Standard - (A2) - M4 x 16:12
- [Mate]: Nyloc Nut - M4:25 ↔ Socket Cap Screw - Standard - (A2) - M4 x 25:13
- [Mate]: Nyloc Nut - M4:26 ↔ Socket Cap Screw - Standard - (A2) - M4 x 25:14
- [Mate]: Nyloc Nut - M4:27 ↔ Socket Cap Screw - Standard - (A2) - M4 x 16:13
- [Mate]: Nyloc Nut - M4:28 ↔ Socket Cap Screw - Standard - (A2) - M4 x 16:14
- [Mate] (18 mm): Nyloc Nut - M4:25 ↔ Socket Cap Screw - Standard - (A2) - M4 x 25:13
- [Mate] (8 mm): Nyloc Nut - M4:28 ↔ Socket Cap Screw - Standard - (A2) - M4 x 16:14
- [Mate] (8 mm): Nyloc Nut - M4:27 ↔ Socket Cap Screw - Standard - (A2) - M4 x 16:13
- [Mate] (18 mm): Nyloc Nut - M4:26 ↔ Socket Cap Screw - Standard - (A2) - M4 x 25:14
- [Mate]: Top_Angle Bracket:7 ↔ Socket Cap Screw - Standard - (A2) - M4 x 25:14
- [Mate]: Top_Angle Bracket:7 ↔ Socket Cap Screw - Standard - (A2) - M4 x 25:14
- [Mate]: Top_Angle Bracket:7 ↔ Socket Cap Screw - Standard - (A2) - M4 x 25:13
- [Mate]: Top_Angle Bracket:7 ↔ Socket Cap Screw - Standard - (A2) - M4 x 25:13
- [Mate]: Top_Angle Bracket:7 ↔ Socket Cap Screw - Standard - (A2) - M4 x 16:13
- [Mate]: Top_Angle Bracket:7 ↔ Socket Cap Screw - Standard - (A2) - M4 x 16:14
- [Mate]: Top_Angle Bracket:7 ↔ Socket Cap Screw - Standard - (A2) - M4 x 16:13
- [Mate]: Top_Angle Bracket:7 ↔ Socket Cap Screw - Standard - (A2) - M4 x 16:14
- [Mate]: Socket Cap Screw - Standard - (A2) - M4 x 25:15 ↔ Nyloc Nut - M4:29
- [Mate]: Socket Cap Screw - Standard - (A2) - M4 x 25:16 ↔ Nyloc Nut - M4:30
- [Mate]: Nyloc Nut - M4:31 ↔ Socket Cap Screw - Standard - (A2) - M4 x 16:15
- [Mate]: Nyloc Nut - M4:32 ↔ Socket Cap Screw - Standard - (A2) - M4 x 16:16
- [Mate] (18 mm): Socket Cap Screw - Standard - (A2) - M4 x 25:15 ↔ Nyloc Nut - M4:29
- [Mate] (8 mm): Nyloc Nut - M4:32 ↔ Socket Cap Screw - Standard - (A2) - M4 x 16:16
- [Mate] (8 mm): Nyloc Nut - M4:31 ↔ Socket Cap Screw - Standard - (A2) - M4 x 16:15
- [Mate] (18 mm): Socket Cap Screw - Standard - (A2) - M4 x 25:16 ↔ Nyloc Nut - M4:30
- [Mate]: Top_Angle Bracket:8 ↔ Socket Cap Screw - Standard - (A2) - M4 x 25:16
- [Mate]: Top_Angle Bracket:8 ↔ Socket Cap Screw - Standard - (A2) - M4 x 25:16
- [Mate]: Socket Cap Screw - Standard - (A2) - M4 x 25:15 ↔ Top_Angle Bracket:8
- [Mate]: Socket Cap Screw - Standard - (A2) - M4 x 25:15 ↔ Top_Angle Bracket:8
- [Mate]: Top_Angle Bracket:8 ↔ Socket Cap Screw - Standard - (A2) - M4 x 16:15
- [Mate]: Socket Cap Screw - Standard - (A2) - M4 x 16:16 ↔ Top_Angle Bracket:8
- [Mate]: Top_Angle Bracket:8 ↔ Socket Cap Screw - Standard - (A2) - M4 x 16:15
- [Mate]: Socket Cap Screw - Standard - (A2) - M4 x 16:16 ↔ Top_Angle Bracket:8
- [Mate]: Socket Cap Screw - Standard - (A2) - M4 x 25:17 ↔ Nyloc Nut - M4:33
- [Mate]: Socket Cap Screw - Standard - (A2) - M4 x 25:18 ↔ Nyloc Nut - M4:34
- [Mate]: Socket Cap Screw - Standard - (A2) - M4 x 16:17 ↔ Nyloc Nut - M4:35
- [Mate]: Socket Cap Screw - Standard - (A2) - M4 x 16:18 ↔ Nyloc Nut - M4:36
- [Mate] (18 mm): Socket Cap Screw - Standard - (A2) - M4 x 25:17 ↔ Nyloc Nut - M4:33
- [Mate] (8 mm): Socket Cap Screw - Standard - (A2) - M4 x 16:18 ↔ Nyloc Nut - M4:36
- [Mate] (8 mm): Socket Cap Screw - Standard - (A2) - M4 x 16:17 ↔ Nyloc Nut - M4:35
- [Mate] (18 mm): Socket Cap Screw - Standard - (A2) - M4 x 25:18 ↔ Nyloc Nut - M4:34
- [Mate]: Socket Cap Screw - Standard - (A2) - M4 x 25:18 ↔ Top_Angle Bracket:9
- [Mate]: Socket Cap Screw - Standard - (A2) - M4 x 25:18 ↔ Top_Angle Bracket:9
- [Mate]: Top_Angle Bracket:9 ↔ Socket Cap Screw - Standard - (A2) - M4 x 25:17
- [Mate]: Top_Angle Bracket:9 ↔ Socket Cap Screw - Standard - (A2) - M4 x 25:17
- [Mate]: Socket Cap Screw - Standard - (A2) - M4 x 16:17 ↔ Top_Angle Bracket:9
- [Mate]: Top_Angle Bracket:9 ↔ Socket Cap Screw - Standard - (A2) - M4 x 16:18
- [Mate]: Socket Cap Screw - Standard - (A2) - M4 x 16:17 ↔ Top_Angle Bracket:9
- [Mate]: Top_Angle Bracket:9 ↔ Socket Cap Screw - Standard - (A2) - M4 x 16:18
- [Mate]: Socket Cap Screw - Standard - (A2) - M4 x 25:19 ↔ Nyloc Nut - M4:37
- [Mate]: Socket Cap Screw - Standard - (A2) - M4 x 25:20 ↔ Nyloc Nut - M4:38
- [Mate]: Nyloc Nut - M4:39 ↔ Socket Cap Screw - Standard - (A2) - M4 x 16:19
- [Mate]: Nyloc Nut - M4:40 ↔ Socket Cap Screw - Standard - (A2) - M4 x 16:20
- [Mate] (18 mm): Socket Cap Screw - Standard - (A2) - M4 x 25:19 ↔ Nyloc Nut - M4:37
- [Mate] (8 mm): Nyloc Nut - M4:40 ↔ Socket Cap Screw - Standard - (A2) - M4 x 16:20
- [Mate] (8 mm): Nyloc Nut - M4:39 ↔ Socket Cap Screw - Standard - (A2) - M4 x 16:19
- [Mate] (18 mm): Socket Cap Screw - Standard - (A2) - M4 x 25:20 ↔ Nyloc Nut - M4:38
- [Mate]: Top_Angle Bracket:10 ↔ Socket Cap Screw - Standard - (A2) - M4 x 25:20
- [Mate]: Top_Angle Bracket:10 ↔ Socket Cap Screw - Standard - (A2) - M4 x 25:20
- [Mate]: Top_Angle Bracket:10 ↔ Socket Cap Screw - Standard - (A2) - M4 x 25:19
- [Mate]: Top_Angle Bracket:10 ↔ Socket Cap Screw - Standard - (A2) - M4 x 25:19
- [Mate]: Top_Angle Bracket:10 ↔ Socket Cap Screw - Standard - (A2) - M4 x 16:19
- [Mate]: Socket Cap Screw - Standard - (A2) - M4 x 16:20 ↔ Top_Angle Bracket:10
- [Mate]: Top_Angle Bracket:10 ↔ Socket Cap Screw - Standard - (A2) - M4 x 16:19
- [Mate]: Socket Cap Screw - Standard - (A2) - M4 x 16:20 ↔ Top_Angle Bracket:10
- [Mate]: Socket Cap Screw - Standard - (A2) - M4 x 25:21 ↔ Nyloc Nut - M4:41
- [Mate]: Socket Cap Screw - Standard - (A2) - M4 x 25:22 ↔ Nyloc Nut - M4:42
- [Mate]: Socket Cap Screw - Standard - (A2) - M4 x 16:21 ↔ Nyloc Nut - M4:43
- [Mate]: Socket Cap Screw - Standard - (A2) - M4 x 16:22 ↔ Nyloc Nut - M4:44
- [Mate] (18 mm): Socket Cap Screw - Standard - (A2) - M4 x 25:21 ↔ Nyloc Nut - M4:41
- [Mate] (8 mm): Socket Cap Screw - Standard - (A2) - M4 x 16:22 ↔ Nyloc Nut - M4:44
- [Mate] (8 mm): Socket Cap Screw - Standard - (A2) - M4 x 16:21 ↔ Nyloc Nut - M4:43
- [Mate] (18 mm): Socket Cap Screw - Standard - (A2) - M4 x 25:22 ↔ Nyloc Nut - M4:42
- [Mate]: Socket Cap Screw - Standard - (A2) - M4 x 25:22 ↔ Top_Angle Bracket:11
- [Mate]: Socket Cap Screw - Standard - (A2) - M4 x 25:22 ↔ Top_Angle Bracket:11
- [Mate]: Top_Angle Bracket:11 ↔ Socket Cap Screw - Standard - (A2) - M4 x 25:21
- [Mate]: Top_Angle Bracket:11 ↔ Socket Cap Screw - Standard - (A2) - M4 x 25:21
- [Mate]: Socket Cap Screw - Standard - (A2) - M4 x 16:21 ↔ Top_Angle Bracket:11
- [Mate]: Top_Angle Bracket:11 ↔ Socket Cap Screw - Standard - (A2) - M4 x 16:22
- [Mate]: Socket Cap Screw - Standard - (A2) - M4 x 16:21 ↔ Top_Angle Bracket:11
- [Mate]: Top_Angle Bracket:11 ↔ Socket Cap Screw - Standard - (A2) - M4 x 16:22
- [Mate]: Nyloc Nut - M4:45 ↔ Socket Cap Screw - Standard - (A2) - M4 x 25:23
- [Mate]: Nyloc Nut - M4:46 ↔ Socket Cap Screw - Standard - (A2) - M4 x 25:24
- [Mate]: Nyloc Nut - M4:47 ↔ Socket Cap Screw - Standard - (A2) - M4 x 16:23
- [Mate]: Nyloc Nut - M4:48 ↔ Socket Cap Screw - Standard - (A2) - M4 x 16:24
- [Mate] (18 mm): Nyloc Nut - M4:45 ↔ Socket Cap Screw - Standard - (A2) - M4 x 25:23
- [Mate] (8 mm): Nyloc Nut - M4:48 ↔ Socket Cap Screw - Standard - (A2) - M4 x 16:24
- [Mate] (8 mm): Nyloc Nut - M4:47 ↔ Socket Cap Screw - Standard - (A2) - M4 x 16:23
- [Mate] (18 mm): Nyloc Nut - M4:46 ↔ Socket Cap Screw - Standard - (A2) - M4 x 25:24
- [Mate]: Top_Angle Bracket:12 ↔ Socket Cap Screw - Standard - (A2) - M4 x 25:24
- [Mate]: Top_Angle Bracket:12 ↔ Socket Cap Screw - Standard - (A2) - M4 x 25:24
- [Mate]: Top_Angle Bracket:12 ↔ Socket Cap Screw - Standard - (A2) - M4 x 25:23
- [Mate]: Top_Angle Bracket:12 ↔ Socket Cap Screw - Standard - (A2) - M4 x 25:23
- [Mate]: Top_Angle Bracket:12 ↔ Socket Cap Screw - Standard - (A2) - M4 x 16:23
- [Mate]: Top_Angle Bracket:12 ↔ Socket Cap Screw - Standard - (A2) - M4 x 16:24
- [Mate]: Top_Angle Bracket:12 ↔ Socket Cap Screw - Standard - (A2) - M4 x 16:23
- [Mate]: Top_Angle Bracket:12 ↔ Socket Cap Screw - Standard - (A2) - M4 x 16:24
- [Mate]: Socket Cap Screw - Standard - (A2) - M4 x 25:25 ↔ Nyloc Nut - M4:49
- [Mate]: Socket Cap Screw - Standard - (A2) - M4 x 25:26 ↔ Nyloc Nut - M4:50
- [Mate]: Nyloc Nut - M4:51 ↔ Socket Cap Screw - Standard - (A2) - M4 x 16:25
- [Mate]: Nyloc Nut - M4:52 ↔ Socket Cap Screw - Standard - (A2) - M4 x 16:26
- [Mate] (18 mm): Socket Cap Screw - Standard - (A2) - M4 x 25:25 ↔ Nyloc Nut - M4:49
- [Mate] (8 mm): Nyloc Nut - M4:52 ↔ Socket Cap Screw - Standard - (A2) - M4 x 16:26
- [Mate] (8 mm): Nyloc Nut - M4:51 ↔ Socket Cap Screw - Standard - (A2) - M4 x 16:25
- [Mate] (18 mm): Socket Cap Screw - Standard - (A2) - M4 x 25:26 ↔ Nyloc Nut - M4:50
- [Mate]: Top_Angle Bracket:13 ↔ Socket Cap Screw - Standard - (A2) - M4 x 25:26
- [Mate]: Top_Angle Bracket:13 ↔ Socket Cap Screw - Standard - (A2) - M4 x 25:26
- [Mate]: Socket Cap Screw - Standard - (A2) - M4 x 25:25 ↔ Top_Angle Bracket:13
- [Mate]: Socket Cap Screw - Standard - (A2) - M4 x 25:25 ↔ Top_Angle Bracket:13
- [Mate]: Top_Angle Bracket:13 ↔ Socket Cap Screw - Standard - (A2) - M4 x 16:25
- [Mate]: Socket Cap Screw - Standard - (A2) - M4 x 16:26 ↔ Top_Angle Bracket:13
- [Mate]: Top_Angle Bracket:13 ↔ Socket Cap Screw - Standard - (A2) - M4 x 16:25
- [Mate]: Socket Cap Screw - Standard - (A2) - M4 x 16:26 ↔ Top_Angle Bracket:13
- [Mate]: Socket Cap Screw - Standard - (A2) - M4 x 25:27 ↔ Nyloc Nut - M4:53
- [Mate]: Socket Cap Screw - Standard - (A2) - M4 x 25:28 ↔ Nyloc Nut - M4:54
- [Mate]: Socket Cap Screw - Standard - (A2) - M4 x 16:27 ↔ Nyloc Nut - M4:55
- [Mate]: Socket Cap Screw - Standard - (A2) - M4 x 16:28 ↔ Nyloc Nut - M4:56
- [Mate] (18 mm): Socket Cap Screw - Standard - (A2) - M4 x 25:27 ↔ Nyloc Nut - M4:53
- [Mate] (8 mm): Socket Cap Screw - Standard - (A2) - M4 x 16:28 ↔ Nyloc Nut - M4:56
- [Mate] (8 mm): Socket Cap Screw - Standard - (A2) - M4 x 16:27 ↔ Nyloc Nut - M4:55
- [Mate] (18 mm): Socket Cap Screw - Standard - (A2) - M4 x 25:28 ↔ Nyloc Nut - M4:54
- [Mate]: Top_Angle Bracket:14 ↔ Socket Cap Screw - Standard - (A2) - M4 x 25:28
- [Mate]: Top_Angle Bracket:14 ↔ Socket Cap Screw - Standard - (A2) - M4 x 25:28
- [Mate]: Top_Angle Bracket:14 ↔ Socket Cap Screw - Standard - (A2) - M4 x 25:27
- [Mate]: Top_Angle Bracket:14 ↔ Socket Cap Screw - Standard - (A2) - M4 x 25:27
- [Mate]: Top_Angle Bracket:14 ↔ Socket Cap Screw - Standard - (A2) - M4 x 16:27
- [Mate]: Top_Angle Bracket:14 ↔ Socket Cap Screw - Standard - (A2) - M4 x 16:28
- [Mate]: Top_Angle Bracket:14 ↔ Socket Cap Screw - Standard - (A2) - M4 x 16:27
- [Mate]: Top_Angle Bracket:14 ↔ Socket Cap Screw - Standard - (A2) - M4 x 16:28
- Mate:320: Top_Backboard:1 ↔ Top_Angle Bracket:1
- Mate:321: Top_Backboard:1 ↔ Socket Cap Screw - Standard - (A2) - M4 x 25:1
- Mate:322: Top_Backboard:1 ↔ Socket Cap Screw - Standard - (A2) - M4 x 25:2
- Mate:323: Top_Backboard:1 ↔ Top_Angle Bracket:2
- Mate:324: Top_Backboard:1 ↔ Top_Angle Bracket:3
- Mate:325: Top_Backboard:1 ↔ Top_Angle Bracket:4
- Mate:326: Top_Backboard:1 ↔ Top_Angle Bracket:5
- Mate:327: Top_Backboard:1 ↔ Top_Angle Bracket:6
- Mate:328: Top_Backboard:1 ↔ Top_Angle Bracket:7
- Mate:329: Top_Backboard:1 ↔ Top_Angle Bracket:8
- Mate:330: Top_Backboard:1 ↔ Top_Angle Bracket:9
- Mate:331: Top_Backboard:1 ↔ Top_Angle Bracket:10
- Mate:332: Top_Backboard:1 ↔ Top_Angle Bracket:11
- Mate:333: Top_Backboard:1 ↔ Top_Angle Bracket:12
- Mate:334: Top_Backboard:1 ↔ Top_Angle Bracket:13
- Mate:335: Top_Backboard:1 ↔ Top_Angle Bracket:14
- Mate:336: Top_Backboard:1 ↔ Socket Cap Screw - Standard - (A2) - M4 x 25:3
- Mate:337: Top_Backboard:1 ↔ Socket Cap Screw - Standard - (A2) - M4 x 25:4
- Mate:338: Top_Backboard:1 ↔ Socket Cap Screw - Standard - (A2) - M4 x 25:5
- Mate:339: Top_Backboard:1 ↔ Socket Cap Screw - Standard - (A2) - M4 x 25:6
- Mate:340: Top_Backboard:1 ↔ Socket Cap Screw - Standard - (A2) - M4 x 25:7
- Mate:341: Top_Backboard:1 ↔ Socket Cap Screw - Standard - (A2) - M4 x 25:8
- Mate:342: Top_Backboard:1 ↔ Socket Cap Screw - Standard - (A2) - M4 x 25:9
- Mate:343: Top_Backboard:1 ↔ Socket Cap Screw - Standard - (A2) - M4 x 25:10
- Mate:344: Top_Backboard:1 ↔ Socket Cap Screw - Standard - (A2) - M4 x 25:11
- Mate:345: Top_Backboard:1 ↔ Socket Cap Screw - Standard - (A2) - M4 x 25:12
- Mate:346: Top_Backboard:1 ↔ Socket Cap Screw - Standard - (A2) - M4 x 25:23
- Mate:347: Top_Backboard:1 ↔ Socket Cap Screw - Standard - (A2) - M4 x 25:24
- Mate:348: Top_Backboard:1 ↔ Socket Cap Screw - Standard - (A2) - M4 x 25:13
- Mate:349: Top_Backboard:1 ↔ Socket Cap Screw - Standard - (A2) - M4 x 25:14
- Mate:350: Top_Backboard:1 ↔ Socket Cap Screw - Standard - (A2) - M4 x 25:15
- Mate:351: Top_Backboard:1 ↔ Socket Cap Screw - Standard - (A2) - M4 x 25:16
- Mate:352: Top_Backboard:1 ↔ Socket Cap Screw - Standard - (A2) - M4 x 25:17
- Mate:353: Top_Backboard:1 ↔ Socket Cap Screw - Standard - (A2) - M4 x 25:18
- Mate:354: Top_Backboard:1 ↔ Socket Cap Screw - Standard - (A2) - M4 x 25:19
- Mate:355: Top_Backboard:1 ↔ Socket Cap Screw - Standard - (A2) - M4 x 25:20
- Mate:356: Top_Backboard:1 ↔ Socket Cap Screw - Standard - (A2) - M4 x 25:21
- Mate:357: Top_Backboard:1 ↔ Socket Cap Screw - Standard - (A2) - M4 x 25:22
- Mate:358: Top_Backboard:1 ↔ Socket Cap Screw - Standard - (A2) - M4 x 25:25
- Mate:359: Top_Backboard:1 ↔ Socket Cap Screw - Standard - (A2) - M4 x 25:26
- Mate:360: Top_Backboard:1 ↔ Socket Cap Screw - Standard - (A2) - M4 x 25:27
- Mate:361: Top_Backboard:1 ↔ Socket Cap Screw - Standard - (A2) - M4 x 25:28
- Mate:362: Top_Backboard:1 ↔ Top_Reinforcement_LHS:1
- Mate:363: Top_Backboard:1 ↔ Top_Reinforcement_RHS:1
- Mate:364: Top_Backboard:1 ↔ Top_Reinforcement 2:2
- Mate:365: Top_Backboard:1 ↔ Top_Reinforcement 2:3
- Mate:366: Top_Backboard:1 ↔ Top_Reinforcement 2:1
- Mate:367: Top_Backboard:1 ↔ Din97 - 4x25 - Steel Wood Screw:1
- Flush:29: Top_Backboard:1 ↔ Din97 - 4x25 - Steel Wood Screw:1
- Mate:368: Top_Backboard:1 ↔ Din97 - 4x25 - Steel Wood Screw:2
- Flush:30: Top_Backboard:1 ↔ Din97 - 4x25 - Steel Wood Screw:2
- Mate:369: Top_Backboard:1 ↔ Din97 - 4x25 - Steel Wood Screw:3
- Mate:370: Top_Backboard:1 ↔ Din97 - 4x25 - Steel Wood Screw:5
- Mate:371: Top_Backboard:1 ↔ Din97 - 4x25 - Steel Wood Screw:4
- Flush:31: Top_Backboard:1 ↔ Din97 - 4x25 - Steel Wood Screw:3
- Flush:32: Top_Backboard:1 ↔ Din97 - 4x25 - Steel Wood Screw:4